# Autodesk Inventor assembly: Assembly
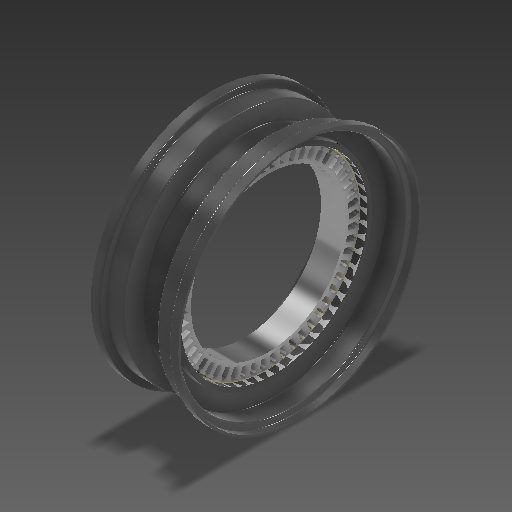
[picture p0: Inventor's stored thumbnail of the model, 512x512]
Saved by Autodesk Inventor 2026.2 (Build 302298000, 298)
## iProperties
Created: 2026-05-19
Part Number: Assembly
Document SubType Name: Assembly
Designer: LENOVO
Author: LENOVO
## Documents named in this file (4)
- D:\Tugas Akhir\Assembly.iam
- D:\Tugas Akhir\stator.ipt
- D:\Tugas Akhir\magnet.ipt
- D:\Tugas Akhir\velg.ipt
## Components (3 placed, 3 different names)
1. stator:1 — Insert:1
2. magnet:1 — Mate:1
3. velg:2 — Mate:1, Insert:1
## Relationships (2: Mate 1, Insert 1)
- Mate:1: magnet:1 ↔ velg:2
- Insert:1 (-42 mm): stator:1 ↔ velg:2
